# Autodesk Inventor assembly: 000.000 - Стенд
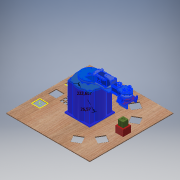
[picture p0: Inventor's stored thumbnail of the model, 180x180]
Saved by Autodesk Inventor 2019 (Build 230136000, 136)
## iProperties
Created: 2020-03-17
Part Number: 000.000 - Стенд
Material: Типовые
Document SubType Name: Assembly
Designer: Петров Иван
Author: Петров Иван
## Documents named in this file (5)
- E:\IVAN\Ivan_desktop\Kvantorium\Competitions\INOP_2020\hardware\SCARA(Dynamixels)\000.000 - Стенд.iam
- E:\IVAN\Ivan_desktop\Kvantorium\Competitions\INOP_2020\hardware\SCARA(Dynamixels)\000.001 - Основание.ipt
- E:\IVAN\Ivan_desktop\Kvantorium\Competitions\INOP_2020\hardware\SCARA(Dynamixels)\000.100 - Манипулятор.iam
- E:\IVAN\Ivan_desktop\Kvantorium\Competitions\INOP_2020\hardware\SCARA(Dynamixels)\000.004 - Куб типа Э (красный).iam
- E:\IVAN\Ivan_desktop\Kvantorium\Competitions\INOP_2020\hardware\SCARA(Dynamixels)\000.008 - Куб типа Ш (зеленый).iam
## Components (4 placed, 4 different names)
1. 000.001 - Основание:1 — Заподлицо:1, Совмещение:3, Совмещение:4, Заподлицо:4, Совмещение:6, Совмещение:7
2. 000.100 - Манипулятор:1 [sub-assembly] — Заподлицо:1, Совмещение:6, Совмещение:7
3. 000.004 - Куб типа Э (красный):1 [sub-assembly] — Совмещение:3, Совмещение:4, Совмещение:5, Заподлицо:2, Заподлицо:3, Заподлицо:4
4. 000.008 - Куб типа Ш (зеленый):1 [sub-assembly] — Совмещение:5, Заподлицо:2, Заподлицо:3
## Relationships (9: Mate 5, Flush 4)
- Заподлицо:1 [Flush]: 000.001 - Основание:1 ↔ 000.100 - Манипулятор:1
- Совмещение:3 [Mate] (1.38 mm): 000.001 - Основание:1 ↔ 000.004 - Куб типа Э (красный):1
- Совмещение:4 [Mate] (1.38 mm): 000.001 - Основание:1 ↔ 000.004 - Куб типа Э (красный):1
- Совмещение:5 [Mate]: 000.004 - Куб типа Э (красный):1 ↔ 000.008 - Куб типа Ш (зеленый):1
- Заподлицо:2 [Flush] (7.9 mm): 000.004 - Куб типа Э (красный):1 ↔ 000.008 - Куб типа Ш (зеленый):1
- Заподлицо:3 [Flush] (7.9 mm): 000.004 - Куб типа Э (красный):1 ↔ 000.008 - Куб типа Ш (зеленый):1
- Заподлицо:4 [Flush]: 000.001 - Основание:1 ↔ 000.004 - Куб типа Э (красный):1
- Совмещение:6 [Mate]: 000.001 - Основание:1 ↔ 000.100 - Манипулятор:1
- Совмещение:7 [Mate]: 000.001 - Основание:1 ↔ 000.100 - Манипулятор:1
